# Autodesk Inventor assembly: Assembly5
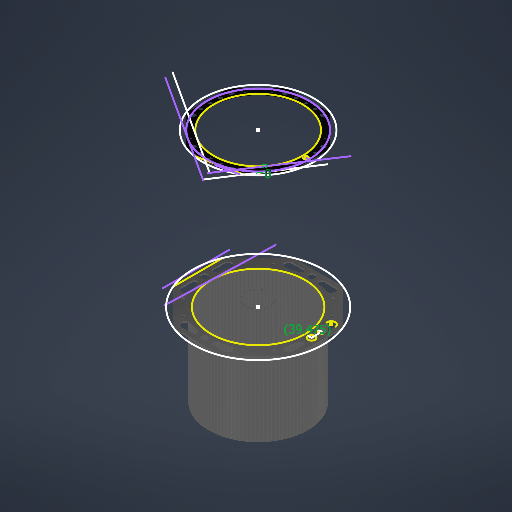
[picture p0: Inventor's stored thumbnail of the model, 512x512]
Saved by Autodesk Inventor 2026.2 (Build 302298000, 298)
## iProperties
Created: 2025-12-11
Part Number: Assembly5
Document SubType Name: Assembly
Designer: Thoma
Author: Thoma
## Documents named in this file (3)
- C:\Users\Thoma\OneDrive\Desktop\Inventor\Quarter_Open\Version_2\Assembly5.iam
- C:\Users\Thoma\OneDrive\Desktop\Inventor\Quarter_Open\Version_2\Telescope_Base.ipt
- C:\Users\Thoma\OneDrive\Desktop\Inventor\Quarter_Open\Version_2\Telescope_End.ipt
## Components (2 placed, 2 different names)
1. Telescope_Base:1 — Angle:1, Mate:1, Mate:2, Angle:2
2. Telescope_End:1 — Angle:1, Mate:1, Mate:2, Angle:2
## Relationships (4: Angle 2, Mate 2)
- Angle:1 (0 deg): Telescope_Base:1 ↔ Telescope_End:1
- Mate:1: Telescope_Base:1 ↔ Telescope_End:1
- Mate:2 (564.023 mm): Telescope_Base:1 ↔ Telescope_End:1
- Angle:2 (0 deg): Telescope_Base:1 ↔ Telescope_End:1
